# Autodesk Inventor assembly: Pancake Piston with Standoffs
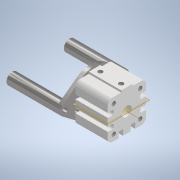
[picture p0: Inventor's stored thumbnail of the model, 180x180]
Saved by Autodesk Inventor 2021 (Build 250183000, 183)
## iProperties
Created: 2021-03-02
Part Number: Pancake Piston with Standoffs
Document SubType Name: Assembly
Designer: aidan
Author: aidan
## Documents named in this file (4)
- C:\Users\aidan\Desktop\T3 Robotics\CAD\Generic and Stock\Pancake Piston with Standoffs.iam
- C:\Users\aidan\Desktop\T3 Robotics\CAD\Generic and Stock\Pancake Shifter.ipt
- C:\Users\aidan\Desktop\T3 Robotics\CAD\Generic and Stock\Pancake Mount Plate.ipt
- C:\Users\aidan\Desktop\T3 Robotics\CAD\Generic and Stock\Piston Mount Standoffs.ipt
## Components (4 placed, 3 different names)
1. Pancake Shifter:1 — Mate:2, Mate:5, Mate:6, Flush:2
2. Pancake Mount Plate:1 — Mate:1, Mate:2, Mate:3, Mate:4, Mate:5, Mate:6
3. Piston Mount Standoffs:1 — Flush:1, Mate:1, Mate:3
4. Piston Mount Standoffs:2 — Flush:1, Mate:4
## Relationships (8: Mate 6, Flush 2)
- Flush:1: Piston Mount Standoffs:1 ↔ Piston Mount Standoffs:2
- Mate:1: Pancake Mount Plate:1 ↔ Piston Mount Standoffs:1
- Mate:2: Pancake Shifter:1 ↔ Pancake Mount Plate:1
- Mate:3: Pancake Mount Plate:1 ↔ Piston Mount Standoffs:1
- Mate:4: Pancake Mount Plate:1 ↔ Piston Mount Standoffs:2
- Mate:5: Pancake Shifter:1 ↔ Pancake Mount Plate:1
- Mate:6: Pancake Shifter:1 ↔ Pancake Mount Plate:1
- Flush:2 (-15.875 mm): Pancake Shifter:1
